# Autodesk Inventor assembly: Monitors_VESA-mountable
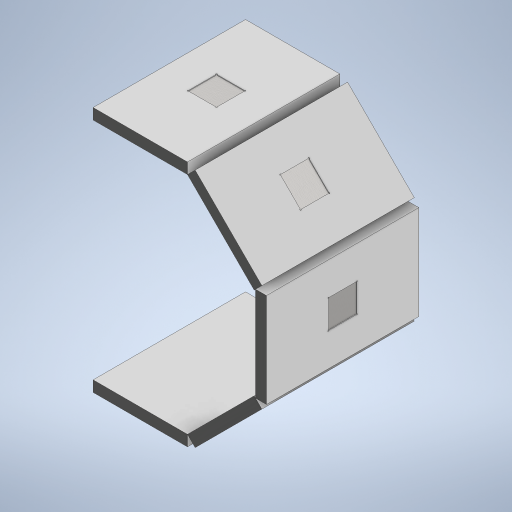
[picture p0: Inventor's stored thumbnail of the model, 512x512]
Saved by Autodesk Inventor 2024 (Build 280153000, 153)
## iProperties
Created: 2023-02-09
Part Number: Monitors_VESA-mountable
Document SubType Name: Assembly
Designer: rosam
Author: rosam
## Documents named in this file (2)
- C:\Users\rosam\OneDrive\Documents\github_latest\Hardware\Tablet-Rig\Assemblies\Monitors_VESA-mountable.iam
- C:\Users\rosam\OneDrive\Documents\github_latest\Hardware\Tablet-Rig\Parts\Monitor-v2.ipt
## Components (5 placed, 1 different names)
1. Monitor-v2:1 — Mate:4, Flush:1, Flush:2, Symmetry:1, Flush:5, Mate:7
2. Monitor-v2:2 — Mate:4, Flush:1, Flush:2, Symmetry:1, Flush:3, Angle:1, Flush:4, Angle:2, Angle:3, Mate:6, Mate:9, Flush:6, Mate:10
3. Monitor-v2:3 — Flush:5, Angle:2, Mate:6
4. Monitor-v2:4 — Flush:4, Angle:3, Mate:7, Mate:8
5. Monitor-v2:5 — Flush:3, Angle:1, Mate:5, Mate:8
## Relationships (17: Mate 7, Flush 6, Angle 3, Symmetry 1)
- Mate:4 (-863.6 mm): Monitor-v2:1 ↔ Monitor-v2:2
- Flush:1: Monitor-v2:1 ↔ Monitor-v2:2
- Flush:2: Monitor-v2:1 ↔ Monitor-v2:2
- Symmetry:1: Monitor-v2:1 ↔ Monitor-v2:2
- Flush:3: Monitor-v2:2 ↔ Monitor-v2:5
- Angle:1 (90 deg): Monitor-v2:2 ↔ Monitor-v2:5
- Mate:5: Monitor-v2:5
- Flush:4: Monitor-v2:2 ↔ Monitor-v2:4
- Flush:5: Monitor-v2:1 ↔ Monitor-v2:3
- Angle:2 (45 deg): Monitor-v2:2 ↔ Monitor-v2:3
- Angle:3 (135 deg): Monitor-v2:2 ↔ Monitor-v2:4
- Mate:6: Monitor-v2:2 ↔ Monitor-v2:3
- Mate:7: Monitor-v2:1 ↔ Monitor-v2:4
- Mate:8: Monitor-v2:4 ↔ Monitor-v2:5
- Mate:9: Monitor-v2:2
- Flush:6: Monitor-v2:2
- Mate:10: Monitor-v2:2
